# Autodesk Inventor assembly: Bearing 608 ASM
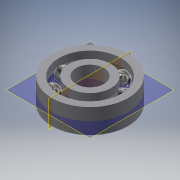
[picture p0: Inventor's stored thumbnail of the model, 180x180]
Saved by Autodesk Inventor 2018 (Build 220112000, 112)
## iProperties
Created: 2017-09-15
Part Number: Bearing 608 ASM
Document SubType Name: Assembly
Designer: Rus
Author: Rus
## Documents named in this file (4)
- E:\Libraries\Documents\3D Models\Bearings\608\Bearing 608 ASM.iam
- E:\Libraries\Documents\3D Models\Bearings\608\Bearing 608 Inner Race.ipt
- E:\Libraries\Documents\3D Models\Bearings\608\Bearing 608 Outer Race.ipt
- E:\Libraries\Documents\3D Models\Bearings\608\Bearing 608 Ball Bearing.ipt
## Components (9 placed, 3 different names)
1. Bearing 608 Inner Race:1 — Flush:1, Mate:1, Mate:2, Symmetry:1
2. Bearing 608 Outer Race:1 — Flush:1, Mate:1, Mate:2, Flush:2, Symmetry:1, Mate:17
3. Bearing 608 Ball Bearing:1 — Mate:15
4. Bearing 608 Ball Bearing:8
5. Bearing 608 Ball Bearing:9
6. Bearing 608 Ball Bearing:10
7. Bearing 608 Ball Bearing:11
8. Bearing 608 Ball Bearing:12
9. Bearing 608 Ball Bearing:13
## Component patterns: (7 elements, first: Bearing 608 Ball Bearing:1)
## Relationships (9: Mate 6, Flush 2, Symmetry 1)
- Flush:1: Bearing 608 Inner Race:1 ↔ Bearing 608 Outer Race:1
- Mate:1: Bearing 608 Inner Race:1 ↔ Bearing 608 Outer Race:1
- Mate:2: Bearing 608 Inner Race:1 ↔ Bearing 608 Outer Race:1
- Flush:2: Bearing 608 Outer Race:1
- Symmetry:1: Bearing 608 Inner Race:1 ↔ Bearing 608 Outer Race:1
- Mate:15: Bearing 608 Ball Bearing:1
- Mate:17: Bearing 608 Outer Race:1
- Mate:18
- Mate:19
